# Autodesk Inventor assembly: 21700PACK
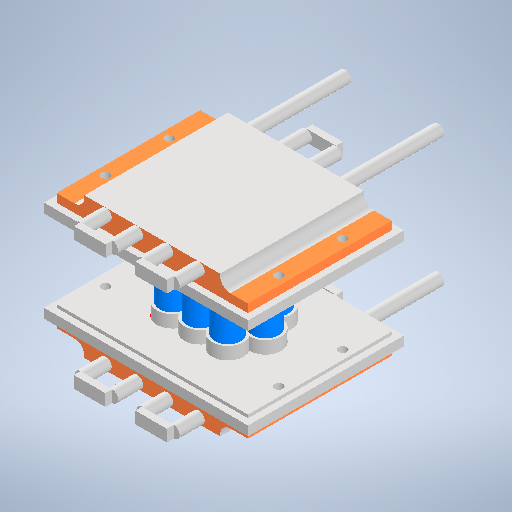
[picture p0: Inventor's stored thumbnail of the model, 512x512]
Saved by Autodesk Inventor 2025.2 (Build 292293000, 293)
## iProperties
Created: 2025-01-16
Part Number: 21700PACK
Document SubType Name: Assembly
Designer: cbast
Author: cbast
## Documents named in this file (6)
- C:\Users\cbast\OneDrive\Documents\21700PACK.iam
- C:\Users\cbast\OneDrive\Documents\21700(Blue).ipt
- C:\Users\cbast\OneDrive\Documents\CELLCASE21700.ipt
- C:\Users\cbast\OneDrive\Documents\nickel strip.ipt
- C:\Users\cbast\OneDrive\Documents\cooling plate.ipt
- C:\Users\cbast\OneDrive\Documents\343thermalpad.ipt
## Components (18 placed, 5 different names)
1. 21700(Blue):1 — Mate:2, Flush:7
2. 21700(Blue):2 — Mate:1, Flush:4
3. 21700(Blue):3 — Mate:3, Flush:10
4. 21700(Blue):4 — Mate:4, Flush:1, Mate:12
5. 21700(Blue):5 — Mate:5, Flush:3
6. 21700(Blue):6 — Mate:10, Flush:8
7. 21700(Blue):7 — Mate:9, Flush:5
8. 21700(Blue):8 — Mate:8, Flush:2
9. 21700(Blue):9 — Mate:7, Flush:9, Mate:11, Flush:11
10. 21700(Blue):10 — Mate:6, Flush:6, Mate:18
11. CELLCASE21700:1 — Mate:1, Mate:2, Mate:3, Mate:4, Mate:5, Mate:6, Mate:7, Mate:8, Mate:9, Mate:10, Flush:1, Flush:2, Flush:3, Flush:4, Flush:5, Flush:6, Flush:7, Flush:8, Flush:9, Flush:10, Mate:13, Mate:16, Mate:17
12. CELLCASE21700:2 — Mate:11, Mate:12, Flush:11, Mate:21, Mate:22
13. nickel strip:1 — Mate:18, Mate:19
14. nickel strip:2 — Mate:13, Mate:14
15. 343thermalpad:1 — Mate:19, Mate:20
16. 343thermalpad:2 — Mate:14, Mate:15
17. cooling plate:1 — Mate:15, Mate:16, Mate:17
18. cooling plate:2 — Mate:20, Mate:21, Mate:22
## Relationships (33: Mate 22, Flush 11)
- Mate:1: 21700(Blue):2 ↔ CELLCASE21700:1
- Mate:2: 21700(Blue):1 ↔ CELLCASE21700:1
- Mate:3: 21700(Blue):3 ↔ CELLCASE21700:1
- Mate:4: 21700(Blue):4 ↔ CELLCASE21700:1
- Mate:5: 21700(Blue):5 ↔ CELLCASE21700:1
- Mate:6: 21700(Blue):10 ↔ CELLCASE21700:1
- Mate:7: 21700(Blue):9 ↔ CELLCASE21700:1
- Mate:8: 21700(Blue):8 ↔ CELLCASE21700:1
- Mate:9: 21700(Blue):7 ↔ CELLCASE21700:1
- Mate:10: 21700(Blue):6 ↔ CELLCASE21700:1
- Flush:1: 21700(Blue):4 ↔ CELLCASE21700:1
- Flush:2: 21700(Blue):8 ↔ CELLCASE21700:1
- Flush:3: 21700(Blue):5 ↔ CELLCASE21700:1
- Flush:4: 21700(Blue):2 ↔ CELLCASE21700:1
- Flush:5: 21700(Blue):7 ↔ CELLCASE21700:1
- Flush:6: 21700(Blue):10 ↔ CELLCASE21700:1
- Flush:7: 21700(Blue):1 ↔ CELLCASE21700:1
- Flush:8: 21700(Blue):6 ↔ CELLCASE21700:1
- Flush:9: 21700(Blue):9 ↔ CELLCASE21700:1
- Flush:10: 21700(Blue):3 ↔ CELLCASE21700:1
- Mate:11: 21700(Blue):9 ↔ CELLCASE21700:2
- Mate:12: 21700(Blue):4 ↔ CELLCASE21700:2
- Flush:11: 21700(Blue):9 ↔ CELLCASE21700:2
- Mate:13: CELLCASE21700:1 ↔ nickel strip:2
- Mate:14: nickel strip:2 ↔ 343thermalpad:2
- Mate:15: 343thermalpad:2 ↔ cooling plate:1
- Mate:16: CELLCASE21700:1 ↔ cooling plate:1
- Mate:17: CELLCASE21700:1 ↔ cooling plate:1
- Mate:18: 21700(Blue):10 ↔ nickel strip:1
- Mate:19: nickel strip:1 ↔ 343thermalpad:1
- Mate:20: 343thermalpad:1 ↔ cooling plate:2
- Mate:21: CELLCASE21700:2 ↔ cooling plate:2
- Mate:22: CELLCASE21700:2 ↔ cooling plate:2
